# Autodesk Inventor assembly: Toughbox-mini
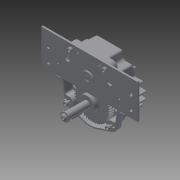
[picture p0: Inventor's stored thumbnail of the model, 180x180]
Saved by Autodesk Inventor 2015 (Build 190159000, 159)
## iProperties
Created: 2015-01-11
Part Number: Toughbox-mini
Document SubType Name: Assembly
Designer: whitaus15
Author: Unknown
Title: S:/Products/Gearboxes Spur Single Stage/Toughbox/Toughbox Mini/Toughbox-Mini.stp
Organization: Unknown
Description: Unknown
Sending System: Unknown
Preprocessor: XStep 1.0
Author: whitaus15
## Documents named in this file (19)
- \\LHSSVR02\Homedirs\Robotics Club\CAD Model 2015\Parts Folder\Gear Boxes\Toughbox-mini.iam
- \\LHSSVR02\Homedirs\Robotics Club\CAD Model 2015\Parts Folder\Gear Boxes\Imported Components\Toughbox-mini\r6zz.ipt
- \\LHSSVR02\Homedirs\Robotics Club\CAD Model 2015\Parts Folder\Gear Boxes\Imported Components\Toughbox-mini\Toughbox_d03.ipt
- \\LHSSVR02\Homedirs\Robotics Club\CAD Model 2015\Parts Folder\Gear Boxes\Imported Components\Toughbox-mini\Toughbox_d07.ipt
- \\LHSSVR02\Homedirs\Robotics Club\CAD Model 2015\Parts Folder\Gear Boxes\Imported Components\Toughbox-mini\Toughbox_d05.ipt
- \\LHSSVR02\Homedirs\Robotics Club\CAD Model 2015\Parts Folder\Gear Boxes\Imported Components\Toughbox-mini\Toughbox_d08.ipt
- \\LHSSVR02\Homedirs\Robotics Club\CAD Model 2015\Parts Folder\Gear Boxes\Imported Components\Toughbox-mini\Toughbox_d06.ipt
- \\LHSSVR02\Homedirs\Robotics Club\CAD Model 2015\Parts Folder\Gear Boxes\Imported Components\Toughbox-mini\fr-6-zz.ipt
- \\LHSSVR02\Homedirs\Robotics Club\CAD Model 2015\Parts Folder\Gear Boxes\Imported Components\Toughbox-mini\fr-8-zz.ipt
- \\LHSSVR02\Homedirs\Robotics Club\CAD Model 2015\Parts Folder\Gear Boxes\Imported Components\Toughbox-mini\10-32_nylock_nut.ipt
- \\LHSSVR02\Homedirs\Robotics Club\CAD Model 2015\Parts Folder\Gear Boxes\Imported Components\Toughbox-mini\5-16_washer.ipt
- \\LHSSVR02\Homedirs\Robotics Club\CAD Model 2015\Parts Folder\Gear Boxes\Imported Components\Toughbox-mini\Toughbox_d09.ipt
- \\LHSSVR02\Homedirs\Robotics Club\CAD Model 2015\Parts Folder\Gear Boxes\Imported Components\Toughbox-mini\8mm_spring_clip.ipt
- \\LHSSVR02\Homedirs\Robotics Club\CAD Model 2015\Parts Folder\Gear Boxes\Imported Components\Toughbox-mini\Toughbox-mini_d01-5-12.ipt
- \\LHSSVR02\Homedirs\Robotics Club\CAD Model 2015\Parts Folder\Gear Boxes\Imported Components\Toughbox-mini\Toughbox-mini_d02.ipt
- \\LHSSVR02\Homedirs\Robotics Club\CAD Model 2015\Parts Folder\Gear Boxes\Imported Components\Toughbox-mini\250_washer.ipt
- \\LHSSVR02\Homedirs\Robotics Club\CAD Model 2015\Parts Folder\Gear Boxes\Imported Components\Toughbox-mini\14-20x0500_bhcs.ipt
- \\LHSSVR02\Homedirs\Robotics Club\CAD Model 2015\Parts Folder\Gear Boxes\Imported Components\Toughbox-mini\125x124x700_key.ipt
- \\LHSSVR02\Homedirs\Robotics Club\CAD Model 2015\Parts Folder\Gear Boxes\Imported Components\Toughbox-mini\10-32x0625_shcs.ipt
## Components (34 placed, 18 different names)
1. r6zz
2. r6zz:1
3. Toughbox_d03
4. Toughbox_d07
5. Toughbox_d05
6. Toughbox_d08
7. Toughbox_d06
8. fr-6-zz
9. fr-8-zz
10. 10-32_nylock_nut
11. 10-32_nylock_nut:1
12. 10-32_nylock_nut:2
13. 10-32_nylock_nut:3
14. 5-16_washer
15. 5-16_washer:1
16. 5-16_washer:2
17. 5-16_washer:3
18. Toughbox_d09
19. Toughbox_d09:1
20. 8mm_spring_clip
21. 8mm_spring_clip:1
22. Toughbox-mini_d01-5-12 — Mate:1
23. Toughbox-mini_d02 — Mate:1, Insert:1, Insert:2
24. 250_washer
25. 14-20x0500_bhcs
26. 125x124x700_key
27. 10-32x0625_shcs
28. 10-32x0625_shcs:1
29. 10-32x0625_shcs:2 — Insert:1
30. 10-32x0625_shcs:3
31. 10-32x0625_shcs:4 — Insert:2
32. 10-32x0625_shcs:5
33. 10-32x0625_shcs:6
34. 10-32x0625_shcs:7
## Relationships (3: Insert 2, Mate 1)
- Mate:1: Toughbox-mini_d01-5-12 ↔ Toughbox-mini_d02
- Insert:1: Toughbox-mini_d02 ↔ 10-32x0625_shcs:2
- Insert:2: Toughbox-mini_d02 ↔ 10-32x0625_shcs:4
